# Autodesk Inventor assembly: draftEndEffector
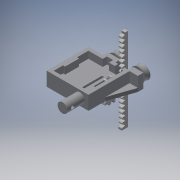
[picture p0: Inventor's stored thumbnail of the model, 180x180]
Saved by Autodesk Inventor 2017 (Build 210142000, 142)
## iProperties
Created: 2018-10-15
Part Number: draftEndEffector
Document SubType Name: Assembly
Designer: Tom
Author: Tom
## Documents named in this file (5)
- C:\Users\Tom\Google Drive\UQ\UNI_WORK\METR4202\Problem Sets\PS3\CAD\draftEndEffector.iam
- C:\Users\Tom\Google Drive\UQ\UNI_WORK\METR4202\Problem Sets\PS3\CAD\Housing.ipt
- C:\Users\Tom\Google Drive\UQ\UNI_WORK\METR4202\Problem Sets\PS3\CAD\Pinion.ipt
- C:\Users\Tom\Google Drive\UQ\UNI_WORK\METR4202\Problem Sets\PS3\CAD\Rack.ipt
- C:\Users\Tom\Google Drive\UQ\UNI_WORK\METR4202\Problem Sets\PS3\CAD\U-Groove-Bearings.ipt
## Components (5 placed, 3 different names)
1. Housing:1 — Angle:1
2. Spur Gear1:1 — Angle:1
3. Spur Gear1:2
4. U-Groove-Bearings:1
5. U-Groove-Bearings:2
## Relationships (1: Angle 1)
- Angle:1 (0 deg): Housing:1 ↔ Spur Gear1:1
